# Autodesk Inventor assembly: Ensemble_Lanceur
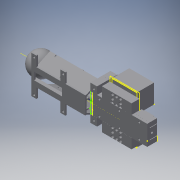
[picture p0: Inventor's stored thumbnail of the model, 180x180]
Saved by Autodesk Inventor 2017 (Build 210142000, 142)
## iProperties
Part Number: Ensemble_Lanceur
Material: Générique
Document SubType Name: Assembly
Designer: Thomas
Author: Thomas
## Documents named in this file (10)
- C:\Users\Thomas\Documents\Modele 3D\Lanceur boule\Ensemble_Lanceur.iam
- C:\Users\Thomas\Documents\Modele 3D\Lanceur boule\cremaillere.ipt
- C:\Users\Thomas\Documents\Modele 3D\Lanceur boule\lanceur.ipt
- C:\Users\Thomas\Documents\Modele 3D\Lanceur boule\support_arret.ipt
- C:\Users\Thomas\Documents\Modele 3D\Lanceur boule\aret.ipt
- C:\Users\Thomas\Documents\Modele 3D\Lanceur boule\percuteur.ipt
- C:\Users\Thomas\Documents\Modele 3D\Lanceur boule\new_cuiller.ipt
- C:\Users\Thomas\Documents\Modele 3D\Lanceur boule\tg.ipt
- C:\Users\Thomas\Documents\Modele 3D\Lanceur boule\Boule.ipt
- C:\Users\Thomas\Documents\Modele 3D\Lanceur boule\Ax12.ipt
## Components (10 placed, 9 different names)
1. cremaillere:1 — Placage:17, Placage:18, Placage:19, Placage:20
2. lanceur:1 — Placage:10, Placage:12, Placage:13, Placage:14, Placage:17
3. aret:1 — Placage:14, Placage:15, Affleurement:1, Placage:18, Affleurement:4, Affleurement:5, Affleurement:6, Placage:27
4. support_arret:1 — Placage:11, Placage:12, Placage:13, Placage:15, Affleurement:1, Placage:21, Placage:22, Placage:23, Placage:24, Placage:25, Placage:26
5. percuteur:1 — Placage:19, Placage:20
6. new_cuiller:1 — Placage:27
7. tg:1 — Affleurement:5, Affleurement:6
8. Boule:1
9. Ax12:2 — Placage:21, Placage:22, Placage:23
10. Ax12:3 — Placage:24, Placage:25, Placage:26
## Relationships (21: Mate 17, Flush 4)
- Placage:10 [Mate]: lanceur:1
- Placage:11 [Mate]: support_arret:1
- Placage:12 [Mate]: lanceur:1 ↔ support_arret:1
- Placage:13 [Mate]: lanceur:1 ↔ support_arret:1
- Placage:14 [Mate]: lanceur:1 ↔ aret:1
- Placage:15 [Mate]: aret:1 ↔ support_arret:1
- Affleurement:1 [Flush]: aret:1 ↔ support_arret:1
- Placage:17 [Mate]: cremaillere:1 ↔ lanceur:1
- Placage:18 [Mate]: cremaillere:1 ↔ aret:1
- Placage:19 [Mate]: cremaillere:1 ↔ percuteur:1
- Placage:20 [Mate]: cremaillere:1 ↔ percuteur:1
- Affleurement:4 [Flush] (100 mm): aret:1
- Affleurement:5 [Flush]: aret:1 ↔ tg:1
- Affleurement:6 [Flush]: aret:1 ↔ tg:1
- Placage:21 [Mate]: support_arret:1 ↔ Ax12:2
- Placage:22 [Mate]: support_arret:1 ↔ Ax12:2
- Placage:23 [Mate]: support_arret:1 ↔ Ax12:2
- Placage:24 [Mate]: support_arret:1 ↔ Ax12:3
- Placage:25 [Mate]: support_arret:1 ↔ Ax12:3
- Placage:26 [Mate]: support_arret:1 ↔ Ax12:3
- Placage:27 [Mate]: aret:1 ↔ new_cuiller:1
